# Autodesk Inventor assembly: Assembly Stepper Motor
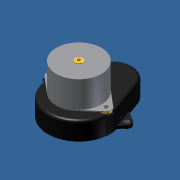
[picture p0: Inventor's stored thumbnail of the model, 180x180]
Saved by Autodesk Inventor 2012 SP1 (Build 160190100, 190)
## iProperties
Created: 2012-06-26
Part Number: Assembly Stepper Motor
Document SubType Name: Assembly
Designer: sta
Author: sta
## Documents named in this file (4)
- R:\Modules\SI\204_PR1 (Kart)\2012\CAD Parts\Motors\Assembly Stepper Motor.iam
- R:\Modules\SI\204_PR1 (Kart)\2012\CAD Parts\Motors\Stepper Motor SAIA Reducer31082011 .ipt
- R:\Modules\SI\204_PR1 (Kart)\2012\CAD Parts\Motors\Stepper Motor SAIA 2012.ipt
- R:\Modules\SI\204_PR1 (Kart)\2012\CAD Parts\Motors\Stepper Motor Rondelle2.ipt
## Components (4 placed, 3 different names)
1. Stepper Motor SAIA Reducer31082011 :1 — Mate:1, Insert:1, Insert:2, Mate:3
2. Stepper Motor SAIA 2012:1 — Mate:1, Mate:2, Mate:3
3. Stepper Motor Rondelle2:1 — Insert:1, Mate:2
4. Stepper Motor Rondelle2:2 — Insert:2
## Relationships (5: Mate 3, Insert 2)
- Mate:1: Stepper Motor SAIA Reducer31082011 :1 ↔ Stepper Motor SAIA 2012:1
- Insert:1: Stepper Motor SAIA Reducer31082011 :1 ↔ Stepper Motor Rondelle2:1
- Insert:2: Stepper Motor SAIA Reducer31082011 :1 ↔ Stepper Motor Rondelle2:2
- Mate:2: Stepper Motor SAIA 2012:1 ↔ Stepper Motor Rondelle2:1
- Mate:3: Stepper Motor SAIA Reducer31082011 :1 ↔ Stepper Motor SAIA 2012:1
